# Autodesk Inventor assembly: inner_mirrored
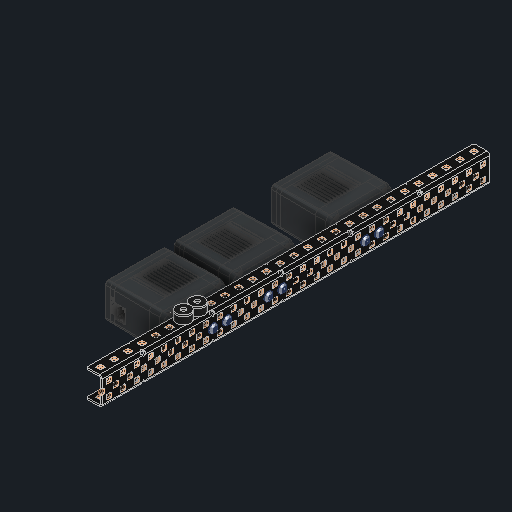
[picture p0: Inventor's stored thumbnail of the model, 512x512]
Saved by Autodesk Inventor 2024 (Build 280153000, 153)
## iProperties
Created: 2024-02-11
Part Number: inner_mirrored
Document SubType Name: Assembly
Designer: Averey Ku
Author: Averey Ku
## Documents named in this file (9)
- D:\vex_robotics\hardware\cad\vroomba_v0.1\chassis\drivebay\mirrored_parts\inner_mirrored.iam
- D:\vex_robotics\hardware\cad\vroomba_v0.1\chassis\drivebay\mirrored_parts\Alu C 1x2x1x28_mirrored.ipt
- D:\vex_robotics\hardware\cad\vroomba_v0.1\chassis\drivebay\mirrored_parts\SteelM-StarS_mirrored.iam
- D:\vex_robotics\hardware\cad\vroomba_v0.1\chassis\drivebay\mirrored_parts\Bearing Flat Low Profile_mirrored.ipt
- D:\vex_robotics\hardware\cad\VEX-CAD-Inventor-1.41\Motion\Spacers\Spacer Nylon .500 OD\NSpacer Black .500 OD x .250.ipt
- D:\vex_robotics\hardware\cad\VEX-CAD-Inventor-1.41\Motion\Spacers\Spacer Nylon .500 OD.ipt
- D:\vex_robotics\hardware\cad\vroomba_v0.1\chassis\drivebay\mirrored_parts\DWasher .500 OD x .062500_mirrored.ipt
- D:\vex_robotics\hardware\cad\vroomba_v0.1\chassis\drivebay\mirrored_parts\Nut Low Profile_mirrored.ipt
- D:\vex_robotics\hardware\cad\vroomba_v0.1\chassis\drivebay\mirrored_parts\1-Post Standoff Retainer_mirrored.ipt
## Components (16 placed, 7 different names)
1. Alu C 1x2x1x28_mirrored:1 — Mate:3, Insert:3, Mate:2, Insert:2, Mate:1, Insert:1, Mate:4, Insert:4, Mate:5, Insert:5, Mate:6, Insert:6, Mate:7, Insert:7, Insert:11, Insert:10, Mate:8, Insert:15, Mate:9, Insert:14
2. SteelM-StarS_mirrored:1 [sub-assembly] — Mate:3, Insert:3
3. SteelM-StarS_mirrored:2 [sub-assembly] — Mate:2, Insert:2
4. SteelM-StarS_mirrored:3 [sub-assembly] — Mate:1, Insert:1
5. Bearing Flat Low Profile_mirrored:1 — Mate:4, Insert:4
6. Bearing Flat Low Profile_mirrored:2 — Mate:5, Insert:5
7. Bearing Flat Low Profile_mirrored:3 — Mate:6, Insert:6
8. Bearing Flat Low Profile_mirrored:4 — Mate:7, Insert:7
9. NSpacer Black .500 OD x .250:1 — Insert:11, Insert:8
10. DWasher .500 OD x .062500_mirrored:1 — Insert:8
11. NSpacer Black .500 OD x .250:2 — Insert:10, Insert:9
12. DWasher .500 OD x .062500_mirrored:2 — Insert:9
13. Nut Low Profile_mirrored:1 — Insert:12
14. 1-Post Standoff Retainer_mirrored:1 — Mate:8, Insert:15, Insert:12
15. Nut Low Profile_mirrored:2 — Insert:13
16. 1-Post Standoff Retainer_mirrored:2 — Mate:9, Insert:14, Insert:13
## Relationships (24: Insert 15, Mate 9)
- Mate:3: Alu C 1x2x1x28_mirrored:1 ↔ SteelM-StarS_mirrored:1
- Insert:3: Alu C 1x2x1x28_mirrored:1 ↔ SteelM-StarS_mirrored:1
- Mate:2: Alu C 1x2x1x28_mirrored:1 ↔ SteelM-StarS_mirrored:2
- Insert:2: Alu C 1x2x1x28_mirrored:1 ↔ SteelM-StarS_mirrored:2
- Mate:1: Alu C 1x2x1x28_mirrored:1 ↔ SteelM-StarS_mirrored:3
- Insert:1: Alu C 1x2x1x28_mirrored:1 ↔ SteelM-StarS_mirrored:3
- Mate:4: Alu C 1x2x1x28_mirrored:1 ↔ Bearing Flat Low Profile_mirrored:1
- Insert:4: Alu C 1x2x1x28_mirrored:1 ↔ Bearing Flat Low Profile_mirrored:1
- Mate:5: Alu C 1x2x1x28_mirrored:1 ↔ Bearing Flat Low Profile_mirrored:2
- Insert:5: Alu C 1x2x1x28_mirrored:1 ↔ Bearing Flat Low Profile_mirrored:2
- Mate:6: Alu C 1x2x1x28_mirrored:1 ↔ Bearing Flat Low Profile_mirrored:3
- Insert:6: Alu C 1x2x1x28_mirrored:1 ↔ Bearing Flat Low Profile_mirrored:3
- Mate:7: Alu C 1x2x1x28_mirrored:1 ↔ Bearing Flat Low Profile_mirrored:4
- Insert:7: Alu C 1x2x1x28_mirrored:1 ↔ Bearing Flat Low Profile_mirrored:4
- Insert:11: Alu C 1x2x1x28_mirrored:1 ↔ NSpacer Black .500 OD x .250:1
- Insert:8: NSpacer Black .500 OD x .250:1 ↔ DWasher .500 OD x .062500_mirrored:1
- Insert:10: Alu C 1x2x1x28_mirrored:1 ↔ NSpacer Black .500 OD x .250:2
- Insert:9: NSpacer Black .500 OD x .250:2 ↔ DWasher .500 OD x .062500_mirrored:2
- Mate:8: Alu C 1x2x1x28_mirrored:1 ↔ 1-Post Standoff Retainer_mirrored:1
- Insert:15: Alu C 1x2x1x28_mirrored:1 ↔ 1-Post Standoff Retainer_mirrored:1
- Insert:12: Nut Low Profile_mirrored:1 ↔ 1-Post Standoff Retainer_mirrored:1
- Mate:9: Alu C 1x2x1x28_mirrored:1 ↔ 1-Post Standoff Retainer_mirrored:2
- Insert:14: Alu C 1x2x1x28_mirrored:1 ↔ 1-Post Standoff Retainer_mirrored:2
- Insert:13: Nut Low Profile_mirrored:2 ↔ 1-Post Standoff Retainer_mirrored:2
